# Autodesk Inventor assembly: Head
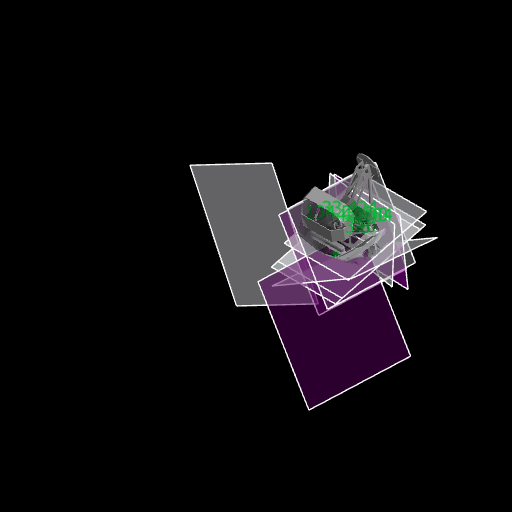
[picture p0: Inventor's stored thumbnail of the model, 512x512]
Saved by Autodesk Inventor 2025.2 (Build 292293000, 293)
## iProperties
Created: 2024-12-17
Part Number: Head
Document SubType Name: Assembly
Designer: valer
Author: valer
## Documents named in this file (42)
- C:\Users\valer\Desktop\str1ker\cad\Head.iam
- C:\Users\valer\Desktop\str1ker\cad\Head.ipt
- C:\Users\valer\Desktop\str1ker\cad\HeadMount.ipt
- C:\Users\valer\Desktop\str1ker\cad\external\DepthSensor\PrimeSenseCarmine1.09.ipt
- C:\Users\valer\Desktop\str1ker\cad\external\HingedThreadedStandoffPart1.ipt
- C:\Users\valer\Desktop\str1ker\cad\external\HingedThreadedStandoffPart2.ipt
- C:\Users\valer\Desktop\str1ker\cad\ShaftD6FemaleCollar.ipt
- C:\Users\valer\Desktop\str1ker\cad\external\ShaftD6-2101-0006-0160.ipt
- C:\Users\valer\Desktop\str1ker\cad\TongueMount.ipt
- C:\Users\valer\Desktop\str1ker\cad\external\SetScrewLiteHub-1308-0016-0006.ipt
- C:\Users\valer\Desktop\str1ker\cad\external\ShaftD6-Short-2101-0006-0020.ipt
- C:\Users\valer\Desktop\str1ker\cad\external\UJoint6D\UJoint6D-Body-4003-1006-1006.ipt
- C:\Users\valer\Desktop\str1ker\cad\external\UJoint6D\UJoint6D-Screw.ipt
- C:\Users\valer\Desktop\str1ker\cad\external\ShaftD6-2100-0006-0200.ipt
- C:\Users\valer\Desktop\str1ker\cad\external\ShaftD6-2101-0006-0140.ipt
- C:\Users\valer\Desktop\str1ker\cad\external\LinearBearing-1612-0612-0035.ipt
- C:\Users\valer\Desktop\str1ker\cad\external\ClampingHub1301-0016-0012.ipt
- C:\Users\valer\Desktop\str1ker\cad\external\ShaftClamp6-6058N14.ipt
- C:\Users\valer\Desktop\str1ker\cad\external\TongueSpeaker.ipt
- C:\Users\valer\Desktop\str1ker\cad\TongueSideLid.ipt
- C:\Users\valer\Desktop\str1ker\cad\TongueSideLidMirror.ipt
- C:\Users\valer\Desktop\str1ker\cad\NoseMount.ipt
- C:\Users\valer\Desktop\str1ker\cad\JawMount.ipt
- C:\Users\valer\Desktop\str1ker\cad\external\93655A703_Male-Female Threaded Hex Standoff.ipt
- C:\Users\valer\Desktop\str1ker\cad\CameraMount.ipt
- C:\Users\valer\Desktop\str1ker\cad\Visor.ipt
- C:\Users\valer\Desktop\str1ker\cad\NeckBase.ipt
- C:\Users\valer\Desktop\str1ker\cad\external\HeadServo\M3RCServoMountBracket.ipt
- C:\Users\valer\Desktop\str1ker\cad\external\NeckActuator\1610-50H-2KG-12V-B07-Body.ipt
- C:\Users\valer\Desktop\str1ker\cad\external\NeckActuator\1610-50H-2KG-12V-B07-Shaft.ipt
- C:\Users\valer\Desktop\str1ker\cad\external\59935K12_Ball Joint Rod End.ipt
- C:\Users\valer\Desktop\str1ker\cad\external\NexusRobot14mmKeywayHub.ipt
- C:\Users\valer\Desktop\str1ker\cad\external\HeadServo\PerfectPass56KG.ipt
- C:\Users\valer\Desktop\str1ker\cad\NeckCover.ipt
- C:\Users\valer\Desktop\str1ker\cad\NeckBracket.ipt
- C:\Users\valer\Desktop\str1ker\cad\NeckBracketMirror.ipt
- C:\Users\valer\Desktop\str1ker\cad\external\4005-0016-0001 Half.iam
- C:\Users\valer\Desktop\str1ker\cad\external\1505-0032-0060.ipt
- C:\Users\valer\Desktop\str1ker\cad\external\1505-0032-0160.ipt
- C:\Users\valer\Desktop\str1ker\cad\external\4005-0016-0001 Ball.ipt
- C:\Users\valer\Desktop\str1ker\cad\external\1221-0032-0002.ipt
- C:\Users\valer\Desktop\str1ker\cad\external\UJoint6D\UJoint6D-CenterDrive-4003-1006-1006.ipt
## Components (87 placed, 41 different names)
1. Head:1 — Flush:1, Flush:2, Mate:1, Flush:3, Mate:4, Mate:5, Mate:6, Mate:7, Mate:8, Mate:9, Mate:10, Mate:11, Mate:12, Mate:13, Mate:14, Mate:15, Mate:16, Mate:17, Mate:18, Mate:19, Mate:20, Mate:59, Angle:13, Mate:89, Mate:90, Flush:13, Mate:119, Mate:121, Flush:15, Flush:16, Flush:17, Flush:18, Flush:19, Mate:124, Mate:125, Mate:126, Mate:127, Mate:128, Mate:129, Flush:20, Mate:131, Mate:132, Mate:133, Flush:157
2. HeadMount:1 — Flush:4, Flush:5, Angle:18, Mate:89, Mate:90, Angle:20, Angle:22, Angle:26, Angle:28, Angle:32, Mate:105, Mate:107, Mate:109, Mate:111, Mate:113, Mate:115, Mate:134, Mate:135, Mate:136, Mate:137, Flush:158, Mate:178, Angle:37, Mate:344, Mate:347, Mate:376, Mate:377, Mate:384, Mate:387, Angle:57, Mate:447, Mate:448, Mate:449, Mate:452, Mate:458, Mate:465, Mate:466, Angle:60, Mate:473
3. PrimeSenseCarmine1.09:1 — Flush:6, Flush:23, Mate:138, Mate:198
4. HingedThreadedStandoffPart1:1 — Mate:4, Mate:5, Mate:25, Mate:26
5. HingedThreadedStandoffPart1:2 — Mate:6, Mate:7, Mate:36, Mate:39
6. HingedThreadedStandoffPart1:3 — Mate:8, Mate:9, Mate:37, Mate:38
7. HingedThreadedStandoffPart1:4 — Mate:10, Mate:11, Mate:23, Mate:24
8. HingedThreadedStandoffPart1:5 — Mate:12, Mate:13, Mate:27, Mate:28
9. HingedThreadedStandoffPart1:6 — Mate:16, Mate:17, Mate:29, Mate:40
10. HingedThreadedStandoffPart1:7 — Mate:14, Mate:15, Mate:30, Mate:31
11. HingedThreadedStandoffPart1:8 — Mate:18, Mate:19, Mate:32, Mate:34
12. HingedThreadedStandoffPart1:9 — Mate:20, Mate:33, Mate:35, Mate:59
13. HingedThreadedStandoffPart2:4 — Mate:23, Mate:24, Flush:7, Flush:8
14. HingedThreadedStandoffPart2:5 — Mate:25, Mate:26, Flush:8, Mate:68
15. HingedThreadedStandoffPart2:6 — Mate:27, Mate:28, Flush:7, Flush:10, Mate:69
16. HingedThreadedStandoffPart2:7 — Mate:29, Mate:40, Mate:45, Mate:47
17. HingedThreadedStandoffPart2:8 — Mate:30, Mate:31, Mate:46, Mate:48
18. HingedThreadedStandoffPart2:9 — Mate:32, Mate:34, Mate:49, Mate:52
19. HingedThreadedStandoffPart2:10 — Mate:33, Mate:35, Mate:50, Mate:51
20. HingedThreadedStandoffPart2:11 — Mate:36, Mate:39, Mate:41, Mate:42
21. HingedThreadedStandoffPart2:12 — Mate:37, Mate:38, Mate:43, Mate:44
22. ShaftD6-2100-0006-0200:1 — Mate:87, Angle:17, Mate:88, Angle:18, Mate:108
23. ShaftD6FemaleCollar:1 — Mate:41, Mate:42, Mate:87, Angle:17, Mate:88
24. ShaftD6FemaleCollar:2 — Mate:43, Mate:44, Mate:91, Mate:92
25. ShaftD6FemaleCollar:3 — Mate:45, Mate:47, Mate:95, Mate:96, Angle:23
26. ShaftD6FemaleCollar:4 — Mate:46, Mate:48, Mate:93, Mate:94, Angle:21
27. ShaftD6FemaleCollar:5 — Mate:49, Mate:52, Mate:99, Mate:100, Angle:30
28. ShaftD6FemaleCollar:6 — Mate:50, Mate:51, Mate:97, Mate:98, Angle:27
29. TongueMount:1 — Mate:66, Mate:67, Angle:11, Mate:68, Mate:69, Mate:71
30. SetScrewLiteHub-1308-0016-0006:1 — Mate:66, Mate:67, Angle:11, Mate:70, Mate:73, Angle:61
31. ShaftD6-Short-2101-0006-0020:1 — Mate:70, Mate:71, Mate:72, Angle:12
32. UJoint6D-Body-4003-1006-1006:1 — Mate:72, Mate:73, Angle:12, Mate:76, Mate:77, Mate:78, Mate:79, Angle:61
33. UJoint6D-Screw:1 — Mate:82, Mate:83
34. UJoint6D-Screw:2 — Mate:76, Mate:77
35. UJoint6D-Screw:3 — Mate:78, Mate:79, Mate:474
36. UJoint6D-Body-4003-1006-1006:2 — Angle:13, Mate:82, Mate:83, Mate:84, Mate:85, Mate:86, Angle:14, Flush:12
37. UJoint6D-Screw:4 — Mate:84, Mate:85, Mate:476
38. ShaftD6-2101-0006-0160:7 — Mate:86, Angle:14, Flush:12, Mate:101, Mate:473, Mate:477, Flush:187
39. ShaftD6-2100-0006-0200:2 — Mate:91, Mate:92, Angle:19, Angle:20, Mate:110
40. ShaftD6-2101-0006-0140:1 — Mate:93, Mate:94, Angle:21, Angle:22, Angle:24, Mate:104
41. ShaftD6-2101-0006-0140:2 — Mate:95, Mate:96, Angle:23, Angle:25, Angle:26, Mate:106
42. ShaftD6-2101-0006-0140:3 — Mate:97, Mate:98, Angle:27, Angle:28, Angle:29, Mate:112
43. ShaftD6-2101-0006-0140:4 — Mate:99, Mate:100, Angle:30, Angle:31, Angle:32, Mate:114
44. LinearBearing-1612-0612-0035:1 — Mate:101, Mate:103, Flush:160
45. ClampingHub1301-0016-0012:1 — Mate:103, Flush:160, Angle:37, Mate:347
46. ShaftClamp6-6058N14:1 — Mate:106, Mate:107
47. ShaftClamp6-6058N14:2 — Mate:104, Mate:105
48. ShaftClamp6-6058N14:3 — Mate:108, Mate:109
49. ShaftClamp6-6058N14:4 — Mate:110, Mate:111
50. ShaftClamp6-6058N14:5 — Mate:114, Mate:115
51. ShaftClamp6-6058N14:6 — Mate:112, Mate:113
52. TongueSpeaker:1 — Mate:119, Mate:122, Mate:123
53. TongueSpeaker:2 — Mate:121, Mate:130
54. TongueSideLid:1 — Mate:124, Mate:125, Mate:126
55. TongueSideLidMirror:1 — Mate:127, Mate:128, Mate:129, Mate:130
56. NoseMount:1 — Flush:21, Mate:131, Mate:132, Mate:133
57. JawMount:1 — Flush:22
58. 93655A703_Male-Female Threaded Hex Standoff:1 — Mate:134, Mate:136, Mate:141, Mate:143
59. 93655A703_Male-Female Threaded Hex Standoff:2 — Mate:135, Mate:137, Mate:142
60. CameraMount:1 — Flush:24, Mate:138, Mate:141, Mate:142, Mate:143, Mate:198
61. Visor:1 — Flush:157, Flush:158, Mate:178
62. M3RCServoMountBracket:1 — Mate:344, Mate:449, Mate:450, Mate:451, Mate:452, Angle:59, Mate:453
63. 1610-50H-2KG-12V-B07-Body:1 — Cylindrical:1, Mate:378, Mate:379, Mate:383
64. 1610-50H-2KG-12V-B07-Shaft:1 — Cylindrical:1, Mate:380, Mate:382, Mate:383
65. 1610-50H-2KG-12V-B07-Body:2 — Mate:385, Mate:386, Mate:390, Mate:391
66. 59935K12_Ball Joint Rod End:1 — Mate:378, Mate:379, Mate:471
67. 59935K12_Ball Joint Rod End:2 — Mate:385, Mate:386, Mate:470
68. 59935K12_Ball Joint Rod End:3 — Mate:376, Mate:380, Mate:382, Mate:384
69. 59935K12_Ball Joint Rod End:4 — Mate:377, Mate:387, Mate:388, Mate:389
70. 1610-50H-2KG-12V-B07-Shaft:2 — Mate:388, Mate:389, Mate:390, Mate:391
71. NexusRobot14mmKeywayHub:1 — Mate:407, Mate:472, Angle:60
72. NeckBase:1 — Mate:407, Angle:57, Mate:434, Mate:458, Mate:472
73. NeckCover:1 — Mate:463, Mate:466, Mate:467
74. NeckBracket:1 — Mate:434, Flush:185, Flush:186, Mate:461, Mate:471
75. NeckBracketMirror:1 — Flush:185, Flush:186, Mate:462, Mate:463, Mate:464, Mate:468, Mate:469, Mate:470
76. 4005-0016-0001 Half:1 [sub-assembly] — Mate:435, Mate:436, Mate:437, Mate:438, Mate:448, Mate:453, Mate:454, Mate:455
77. 1505-0032-0060:1 — Mate:435, Mate:436, Mate:437, Mate:439, Mate:440
78. 1505-0032-0160:1 — Mate:438, Mate:439, Mate:440, Mate:447
79. 4005-0016-0001 Half:2 [sub-assembly] — Mate:456, Mate:457
80. 1505-0032-0060:2
81. 1505-0032-0160:2 — Mate:459, Mate:460
82. PerfectPass56KG:1 — Mate:450, Mate:451, Angle:59
83. 4005-0016-0001 Ball:1 — Mate:454, Mate:455, Mate:456, Mate:457
84. 1221-0032-0002:1 — Mate:459, Mate:460, Mate:461, Mate:462, Mate:468, Mate:469
85. NeckCover:2 — Mate:464, Mate:465, Mate:467
86. UJoint6D-CenterDrive-4003-1006-1006:1 — Mate:474, Mate:476
87. ShaftClamp6-6058N14:7 — Mate:477, Flush:187
## Relationships (234: Mate 179, Flush 27, Angle 25, Symmetry 2, CylindricalJoint 1)
- Flush:1: Head:1
- Flush:2: Head:1
- Mate:1: Head:1
- Flush:3: Head:1
- Flush:4: HeadMount:1
- Flush:5: HeadMount:1
- Flush:6: PrimeSenseCarmine1.09:1
- Mate:4: Head:1 ↔ HingedThreadedStandoffPart1:1
- Mate:5: Head:1 ↔ HingedThreadedStandoffPart1:1
- Mate:6: Head:1 ↔ HingedThreadedStandoffPart1:2
- Mate:7: Head:1 ↔ HingedThreadedStandoffPart1:2
- Mate:8: Head:1 ↔ HingedThreadedStandoffPart1:3
- Mate:9: Head:1 ↔ HingedThreadedStandoffPart1:3
- Mate:10: Head:1 ↔ HingedThreadedStandoffPart1:4
- Mate:11: Head:1 ↔ HingedThreadedStandoffPart1:4
- Mate:12: Head:1 ↔ HingedThreadedStandoffPart1:5
- Mate:13: Head:1 ↔ HingedThreadedStandoffPart1:5
- Mate:14: Head:1 ↔ HingedThreadedStandoffPart1:7
- Mate:15: Head:1 ↔ HingedThreadedStandoffPart1:7
- Mate:16: Head:1 ↔ HingedThreadedStandoffPart1:6
- Mate:17: Head:1 ↔ HingedThreadedStandoffPart1:6
- Mate:18: Head:1 ↔ HingedThreadedStandoffPart1:8
- Mate:19: Head:1 ↔ HingedThreadedStandoffPart1:8
- Mate:20: Head:1 ↔ HingedThreadedStandoffPart1:9
- Mate:23: HingedThreadedStandoffPart1:4 ↔ HingedThreadedStandoffPart2:4
- Mate:24: HingedThreadedStandoffPart1:4 ↔ HingedThreadedStandoffPart2:4
- Mate:25: HingedThreadedStandoffPart1:1 ↔ HingedThreadedStandoffPart2:5
- Mate:26: HingedThreadedStandoffPart1:1 ↔ HingedThreadedStandoffPart2:5
- Mate:27: HingedThreadedStandoffPart1:5 ↔ HingedThreadedStandoffPart2:6
- Mate:28: HingedThreadedStandoffPart1:5 ↔ HingedThreadedStandoffPart2:6
- Mate:29: HingedThreadedStandoffPart1:6 ↔ HingedThreadedStandoffPart2:7
- Mate:30: HingedThreadedStandoffPart1:7 ↔ HingedThreadedStandoffPart2:8
- Mate:31: HingedThreadedStandoffPart1:7 ↔ HingedThreadedStandoffPart2:8
- Mate:32: HingedThreadedStandoffPart1:8 ↔ HingedThreadedStandoffPart2:9
- Mate:33: HingedThreadedStandoffPart1:9 ↔ HingedThreadedStandoffPart2:10
- Mate:34: HingedThreadedStandoffPart1:8 ↔ HingedThreadedStandoffPart2:9
- Mate:35: HingedThreadedStandoffPart1:9 ↔ HingedThreadedStandoffPart2:10
- Mate:36: HingedThreadedStandoffPart1:2 ↔ HingedThreadedStandoffPart2:11
- Mate:37: HingedThreadedStandoffPart1:3 ↔ HingedThreadedStandoffPart2:12
- Mate:38: HingedThreadedStandoffPart1:3 ↔ HingedThreadedStandoffPart2:12
- Mate:39: HingedThreadedStandoffPart1:2 ↔ HingedThreadedStandoffPart2:11
- Mate:40: HingedThreadedStandoffPart1:6 ↔ HingedThreadedStandoffPart2:7
- Flush:7: HingedThreadedStandoffPart2:4 ↔ HingedThreadedStandoffPart2:6
- Flush:8: HingedThreadedStandoffPart2:4 ↔ HingedThreadedStandoffPart2:5
- Mate:41: HingedThreadedStandoffPart2:11 ↔ ShaftD6FemaleCollar:1
- Mate:42: HingedThreadedStandoffPart2:11 ↔ ShaftD6FemaleCollar:1
- Mate:43: HingedThreadedStandoffPart2:12 ↔ ShaftD6FemaleCollar:2
- Mate:44: HingedThreadedStandoffPart2:12 ↔ ShaftD6FemaleCollar:2
- Mate:45: HingedThreadedStandoffPart2:7 ↔ ShaftD6FemaleCollar:3
- Mate:46: HingedThreadedStandoffPart2:8 ↔ ShaftD6FemaleCollar:4
- Mate:47: HingedThreadedStandoffPart2:7 ↔ ShaftD6FemaleCollar:3
- Mate:48: HingedThreadedStandoffPart2:8 ↔ ShaftD6FemaleCollar:4
- Mate:49: HingedThreadedStandoffPart2:9 ↔ ShaftD6FemaleCollar:5
- Mate:50: HingedThreadedStandoffPart2:10 ↔ ShaftD6FemaleCollar:6
- Mate:51: HingedThreadedStandoffPart2:10 ↔ ShaftD6FemaleCollar:6
- Mate:52: HingedThreadedStandoffPart2:9 ↔ ShaftD6FemaleCollar:5
- Mate:59: Head:1 ↔ HingedThreadedStandoffPart1:9
- Flush:10: HingedThreadedStandoffPart2:6
- Mate:66: TongueMount:1 ↔ SetScrewLiteHub-1308-0016-0006:1
- Mate:67: TongueMount:1 ↔ SetScrewLiteHub-1308-0016-0006:1
- Angle:11 (0 deg): TongueMount:1 ↔ SetScrewLiteHub-1308-0016-0006:1
- Mate:68: HingedThreadedStandoffPart2:5 ↔ TongueMount:1
- Mate:69: HingedThreadedStandoffPart2:6 ↔ TongueMount:1
- Mate:70: SetScrewLiteHub-1308-0016-0006:1 ↔ ShaftD6-Short-2101-0006-0020:1
- Mate:71: TongueMount:1 ↔ ShaftD6-Short-2101-0006-0020:1
- Mate:72: ShaftD6-Short-2101-0006-0020:1 ↔ UJoint6D-Body-4003-1006-1006:1
- Mate:73: SetScrewLiteHub-1308-0016-0006:1 ↔ UJoint6D-Body-4003-1006-1006:1
- Angle:12 (0 deg): ShaftD6-Short-2101-0006-0020:1 ↔ UJoint6D-Body-4003-1006-1006:1
- Mate:76: UJoint6D-Body-4003-1006-1006:1 ↔ UJoint6D-Screw:2
- Mate:77: UJoint6D-Body-4003-1006-1006:1 ↔ UJoint6D-Screw:2
- Mate:78: UJoint6D-Body-4003-1006-1006:1 ↔ UJoint6D-Screw:3
- Mate:79: UJoint6D-Body-4003-1006-1006:1 ↔ UJoint6D-Screw:3
- Angle:13 (0 deg): Head:1 ↔ UJoint6D-Body-4003-1006-1006:2
- Mate:82: UJoint6D-Screw:1 ↔ UJoint6D-Body-4003-1006-1006:2
- Mate:83: UJoint6D-Screw:1 ↔ UJoint6D-Body-4003-1006-1006:2
- Mate:84: UJoint6D-Body-4003-1006-1006:2 ↔ UJoint6D-Screw:4
- Mate:85: UJoint6D-Body-4003-1006-1006:2 ↔ UJoint6D-Screw:4
- Mate:86: UJoint6D-Body-4003-1006-1006:2 ↔ ShaftD6-2101-0006-0160:7
- Angle:14 (180 deg): UJoint6D-Body-4003-1006-1006:2 ↔ ShaftD6-2101-0006-0160:7
- Flush:12: UJoint6D-Body-4003-1006-1006:2 ↔ ShaftD6-2101-0006-0160:7
- Mate:87: ShaftD6-2100-0006-0200:1 ↔ ShaftD6FemaleCollar:1
- Angle:17 (0 deg): ShaftD6-2100-0006-0200:1 ↔ ShaftD6FemaleCollar:1
- Mate:88: ShaftD6-2100-0006-0200:1 ↔ ShaftD6FemaleCollar:1
- Angle:18 (0 deg): HeadMount:1 ↔ ShaftD6-2100-0006-0200:1
- Mate:89: Head:1 ↔ HeadMount:1
- Mate:90: Head:1 ↔ HeadMount:1
- Mate:91: ShaftD6FemaleCollar:2 ↔ ShaftD6-2100-0006-0200:2
- Mate:92: ShaftD6FemaleCollar:2 ↔ ShaftD6-2100-0006-0200:2
- Angle:19 (0 deg): ShaftD6-2100-0006-0200:2
- Angle:20 (0 deg): HeadMount:1 ↔ ShaftD6-2100-0006-0200:2
- Mate:93: ShaftD6FemaleCollar:4 ↔ ShaftD6-2101-0006-0140:1
- Mate:94: ShaftD6FemaleCollar:4 ↔ ShaftD6-2101-0006-0140:1
- Angle:21 (0 deg): ShaftD6FemaleCollar:4 ↔ ShaftD6-2101-0006-0140:1
- Angle:22 (0 deg): HeadMount:1 ↔ ShaftD6-2101-0006-0140:1
- Mate:95: ShaftD6FemaleCollar:3 ↔ ShaftD6-2101-0006-0140:2
- Mate:96: ShaftD6FemaleCollar:3 ↔ ShaftD6-2101-0006-0140:2
- Angle:23 (0 deg): ShaftD6FemaleCollar:3 ↔ ShaftD6-2101-0006-0140:2
- Angle:24 (180 deg): ShaftD6-2101-0006-0140:1
- Angle:25 (180 deg): ShaftD6-2101-0006-0140:2
- Angle:26 (0 deg): HeadMount:1 ↔ ShaftD6-2101-0006-0140:2
- Mate:97: ShaftD6FemaleCollar:6 ↔ ShaftD6-2101-0006-0140:3
- Mate:98: ShaftD6FemaleCollar:6 ↔ ShaftD6-2101-0006-0140:3
- Angle:27 (0 deg): ShaftD6FemaleCollar:6 ↔ ShaftD6-2101-0006-0140:3
- Angle:28 (0 deg): HeadMount:1 ↔ ShaftD6-2101-0006-0140:3
- Angle:29 (0 deg): ShaftD6-2101-0006-0140:3
- Mate:99: ShaftD6FemaleCollar:5 ↔ ShaftD6-2101-0006-0140:4
- Mate:100: ShaftD6FemaleCollar:5 ↔ ShaftD6-2101-0006-0140:4
- Angle:30 (0 deg): ShaftD6FemaleCollar:5 ↔ ShaftD6-2101-0006-0140:4
- Angle:31 (0 deg): ShaftD6-2101-0006-0140:4
- Angle:32 (0 deg): HeadMount:1 ↔ ShaftD6-2101-0006-0140:4
- Mate:101: ShaftD6-2101-0006-0160:7 ↔ LinearBearing-1612-0612-0035:1
- Mate:103: LinearBearing-1612-0612-0035:1 ↔ ClampingHub1301-0016-0012:1
- Mate:104: ShaftD6-2101-0006-0140:1 ↔ ShaftClamp6-6058N14:2
- Mate:105: HeadMount:1 ↔ ShaftClamp6-6058N14:2
- Mate:106: ShaftD6-2101-0006-0140:2 ↔ ShaftClamp6-6058N14:1
- Mate:107: HeadMount:1 ↔ ShaftClamp6-6058N14:1
- Mate:108: ShaftD6-2100-0006-0200:1 ↔ ShaftClamp6-6058N14:3
- Mate:109: HeadMount:1 ↔ ShaftClamp6-6058N14:3
- Mate:110: ShaftD6-2100-0006-0200:2 ↔ ShaftClamp6-6058N14:4
- Mate:111: HeadMount:1 ↔ ShaftClamp6-6058N14:4
- Mate:112: ShaftD6-2101-0006-0140:3 ↔ ShaftClamp6-6058N14:6
- Mate:113: HeadMount:1 ↔ ShaftClamp6-6058N14:6
- Mate:114: ShaftD6-2101-0006-0140:4 ↔ ShaftClamp6-6058N14:5
- Mate:115: HeadMount:1 ↔ ShaftClamp6-6058N14:5
- Flush:13: Head:1
- Mate:119: Head:1 ↔ TongueSpeaker:1
- Mate:121: Head:1 ↔ TongueSpeaker:2
- Flush:15: Head:1
- Flush:16: Head:1
- Symmetry:1
- Mate:122: TongueSpeaker:1
- Flush:17: Head:1
- Flush:18: Head:1
- Symmetry:2
- Mate:123: TongueSpeaker:1
- Flush:19: Head:1
- Mate:124: Head:1 ↔ TongueSideLid:1
- Mate:125: Head:1 ↔ TongueSideLid:1
- Mate:126: Head:1 ↔ TongueSideLid:1
- Mate:127: Head:1 ↔ TongueSideLidMirror:1
- Mate:128: Head:1 ↔ TongueSideLidMirror:1
- Mate:129: Head:1 ↔ TongueSideLidMirror:1
- Mate:130: TongueSpeaker:2 ↔ TongueSideLidMirror:1
- Flush:20: Head:1
- Flush:21: NoseMount:1
- Mate:131: Head:1 ↔ NoseMount:1
- Mate:132: Head:1 ↔ NoseMount:1
- Mate:133: Head:1 ↔ NoseMount:1
- Flush:22: JawMount:1
- Mate:134: HeadMount:1 ↔ 93655A703_Male-Female Threaded Hex Standoff:1
- Mate:135: HeadMount:1 ↔ 93655A703_Male-Female Threaded Hex Standoff:2
- Mate:136: HeadMount:1 ↔ 93655A703_Male-Female Threaded Hex Standoff:1
- Mate:137: HeadMount:1 ↔ 93655A703_Male-Female Threaded Hex Standoff:2
- Flush:23: PrimeSenseCarmine1.09:1
- Flush:24: CameraMount:1
- Mate:138: PrimeSenseCarmine1.09:1 ↔ CameraMount:1
- Mate:141: 93655A703_Male-Female Threaded Hex Standoff:1 ↔ CameraMount:1
- Mate:142: 93655A703_Male-Female Threaded Hex Standoff:2 ↔ CameraMount:1
- Mate:143: 93655A703_Male-Female Threaded Hex Standoff:1 ↔ CameraMount:1
- Flush:157: Head:1 ↔ Visor:1
- Flush:158: HeadMount:1 ↔ Visor:1
- Mate:178: HeadMount:1 ↔ Visor:1
- Flush:160: LinearBearing-1612-0612-0035:1 ↔ ClampingHub1301-0016-0012:1
- Mate:198: PrimeSenseCarmine1.09:1 ↔ CameraMount:1
- Angle:37 (0 deg): HeadMount:1 ↔ ClampingHub1301-0016-0012:1
- Mate:344: HeadMount:1 ↔ M3RCServoMountBracket:1
- Mate:347: HeadMount:1 ↔ ClampingHub1301-0016-0012:1
- Mate:376: HeadMount:1 ↔ 59935K12_Ball Joint Rod End:3
- Mate:377: HeadMount:1 ↔ 59935K12_Ball Joint Rod End:4
- Cylindrical:1: 1610-50H-2KG-12V-B07-Body:1 ↔ 1610-50H-2KG-12V-B07-Shaft:1
- Mate:378: 1610-50H-2KG-12V-B07-Body:1 ↔ 59935K12_Ball Joint Rod End:1
- Mate:379: 1610-50H-2KG-12V-B07-Body:1 ↔ 59935K12_Ball Joint Rod End:1
- Mate:380: 1610-50H-2KG-12V-B07-Shaft:1 ↔ 59935K12_Ball Joint Rod End:3
- Mate:382: 1610-50H-2KG-12V-B07-Shaft:1 ↔ 59935K12_Ball Joint Rod End:3
- Mate:383: 1610-50H-2KG-12V-B07-Body:1 ↔ 1610-50H-2KG-12V-B07-Shaft:1
- Mate:384 (8 mm): HeadMount:1 ↔ 59935K12_Ball Joint Rod End:3
- Mate:385: 1610-50H-2KG-12V-B07-Body:2 ↔ 59935K12_Ball Joint Rod End:2
- Mate:386: 1610-50H-2KG-12V-B07-Body:2 ↔ 59935K12_Ball Joint Rod End:2
- Mate:387 (8 mm): HeadMount:1 ↔ 59935K12_Ball Joint Rod End:4
- Mate:388: 59935K12_Ball Joint Rod End:4 ↔ 1610-50H-2KG-12V-B07-Shaft:2
- Mate:389: 59935K12_Ball Joint Rod End:4 ↔ 1610-50H-2KG-12V-B07-Shaft:2
- Mate:390: 1610-50H-2KG-12V-B07-Body:2 ↔ 1610-50H-2KG-12V-B07-Shaft:2
- Mate:391: 1610-50H-2KG-12V-B07-Body:2 ↔ 1610-50H-2KG-12V-B07-Shaft:2
- Mate:407: NexusRobot14mmKeywayHub:1 ↔ NeckBase:1
- Angle:57 (0 deg): HeadMount:1 ↔ NeckBase:1
- Mate:434: NeckBase:1 ↔ NeckBracket:1
- Flush:185: NeckBracket:1 ↔ NeckBracketMirror:1
- Flush:186: NeckBracket:1 ↔ NeckBracketMirror:1
- Mate:435: 4005-0016-0001 Half:1 ↔ 1505-0032-0060:1
- Mate:436: 4005-0016-0001 Half:1 ↔ 1505-0032-0060:1
- Mate:437: 4005-0016-0001 Half:1 ↔ 1505-0032-0060:1
- Mate:438: 4005-0016-0001 Half:1 ↔ 1505-0032-0160:1
- Mate:439: 1505-0032-0060:1 ↔ 1505-0032-0160:1
- Mate:440: 1505-0032-0060:1 ↔ 1505-0032-0160:1
- [Mate]: 4005-0016-0001 Half:2 ↔ 1505-0032-0060:2
- [Mate]: 4005-0016-0001 Half:2 ↔ 1505-0032-0060:2
- [Mate]: 4005-0016-0001 Half:2 ↔ 1505-0032-0060:2
- [Mate]: 4005-0016-0001 Half:2 ↔ 1505-0032-0160:2
- [Mate]: 1505-0032-0060:2 ↔ 1505-0032-0160:2
- [Mate]: 1505-0032-0060:2 ↔ 1505-0032-0160:2
- Mate:447: HeadMount:1 ↔ 1505-0032-0160:1
- Mate:448: HeadMount:1 ↔ 4005-0016-0001 Half:1
- Mate:449: HeadMount:1 ↔ M3RCServoMountBracket:1
- Mate:450: M3RCServoMountBracket:1 ↔ PerfectPass56KG:1
- Mate:451: M3RCServoMountBracket:1 ↔ PerfectPass56KG:1
- Mate:452: HeadMount:1 ↔ M3RCServoMountBracket:1
- Angle:59 (0 deg): M3RCServoMountBracket:1 ↔ PerfectPass56KG:1
- Mate:453 (13 mm): M3RCServoMountBracket:1 ↔ 4005-0016-0001 Half:1
- Mate:454: 4005-0016-0001 Half:1 ↔ 4005-0016-0001 Ball:1
- Mate:455 (0.25 mm): 4005-0016-0001 Half:1 ↔ 4005-0016-0001 Ball:1
- Mate:456: 4005-0016-0001 Half:2 ↔ 4005-0016-0001 Ball:1
- Mate:457 (0.25 mm): 4005-0016-0001 Half:2 ↔ 4005-0016-0001 Ball:1
- Mate:458: HeadMount:1 ↔ NeckBase:1
- Mate:459: 1505-0032-0160:2 ↔ 1221-0032-0002:1
- Mate:460: 1505-0032-0160:2 ↔ 1221-0032-0002:1
- Mate:461: NeckBracket:1 ↔ 1221-0032-0002:1
- Mate:462: NeckBracketMirror:1 ↔ 1221-0032-0002:1
- Mate:463: NeckCover:1 ↔ NeckBracketMirror:1
- Mate:464: NeckBracketMirror:1 ↔ NeckCover:2
- Mate:465: HeadMount:1 ↔ NeckCover:2
- Mate:466: HeadMount:1 ↔ NeckCover:1
- Mate:467: NeckCover:1 ↔ NeckCover:2
- Mate:468: NeckBracketMirror:1 ↔ 1221-0032-0002:1
- Mate:469: NeckBracketMirror:1 ↔ 1221-0032-0002:1
- Mate:470: 59935K12_Ball Joint Rod End:2 ↔ NeckBracketMirror:1
- Mate:471: 59935K12_Ball Joint Rod End:1 ↔ NeckBracket:1
- Mate:472: NexusRobot14mmKeywayHub:1 ↔ NeckBase:1
- Angle:60 (0 deg): HeadMount:1 ↔ NexusRobot14mmKeywayHub:1
- Mate:473: HeadMount:1 ↔ ShaftD6-2101-0006-0160:7
- Mate:474: UJoint6D-Screw:3 ↔ UJoint6D-CenterDrive-4003-1006-1006:1
- Mate:476: UJoint6D-Screw:4 ↔ UJoint6D-CenterDrive-4003-1006-1006:1
- Mate:477: ShaftD6-2101-0006-0160:7 ↔ ShaftClamp6-6058N14:7
- Flush:187 (2 mm): ShaftD6-2101-0006-0160:7 ↔ ShaftClamp6-6058N14:7
- Angle:61 (0 deg): SetScrewLiteHub-1308-0016-0006:1 ↔ UJoint6D-Body-4003-1006-1006:1
## Named parameters: d829_d821 = 0 mm, d830_d822 = 0 mm, d831_d823 = 0 mm, d832_d824 = 0 mm, d833_d825 = 0 mm, d834_d826 = 0 mm
